# Autodesk Inventor assembly: Raspberry Pi 4 Wall mount
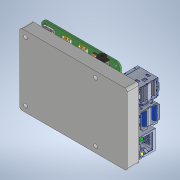
[picture p0: Inventor's stored thumbnail of the model, 180x180]
Saved by Autodesk Inventor 2020.3 (Build 243373010, 373A)
## iProperties
Created: 2021-08-29
Part Number: Raspberry Pi 4 Wall mount
Document SubType Name: Assembly
Designer: Parker
Author: Parker
## Documents named in this file (4)
- D:\Designs\MK3PRO P1\ELECTRONICS\Raspberry Pi 4 Wall mount.iam
- D:\Designs\MK3PRO P1\ELECTRONICS\Raspberry Pi 4\Raspberry Pi 4 Model B.iam
- D:\Designs\MK3PRO P1\ELECTRONICS\Raspberry Pi 4\PoE HAT pi3 b+.ipt
- D:\Designs\MK3PRO P1\ELECTRONICS\Raspberry Pi 4\Pi Back Mount.ipt
## Components (3 placed, 3 different names)
1. Raspberry Pi 4 Model B:1 [sub-assembly] — Mate:1, Mate:2, Mate:3, Mate:4, Mate:5, Mate:6
2. PoE HAT pi3 b+:1 — Mate:1, Mate:2, Mate:3
3. Pi Back Mount:1 — Mate:4, Mate:5, Mate:6
## Relationships (6: Mate 6)
- Mate:1 (7 mm): Raspberry Pi 4 Model B:1 ↔ PoE HAT pi3 b+:1
- Mate:2: Raspberry Pi 4 Model B:1 ↔ PoE HAT pi3 b+:1
- Mate:3: Raspberry Pi 4 Model B:1 ↔ PoE HAT pi3 b+:1
- Mate:4: Raspberry Pi 4 Model B:1 ↔ Pi Back Mount:1
- Mate:5: Raspberry Pi 4 Model B:1 ↔ Pi Back Mount:1
- Mate:6: Raspberry Pi 4 Model B:1 ↔ Pi Back Mount:1
